# Autodesk Inventor assembly: climber assssssembly
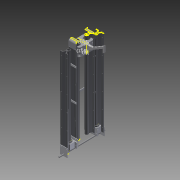
[picture p0: Inventor's stored thumbnail of the model, 180x180]
Saved by Autodesk Inventor 2013 (Build 170138000, 138)
## iProperties
Created: 2013-01-24
Part Number: climber assssssembly
Document SubType Name: Assembly
Designer: Arpan
Mass: 2447.33 g
Surface Area: 6955.59 cm^2
Volume: 1769.33 cm^3
Density: 1.3832 g/cm^3
Author: Arpan
## Documents named in this file (10)
- C:\Users\Arpan\Documents\GitHub\frc2013CAD\Climber\climber assssssembly.iam
- C:\Users\Arpan\Documents\GitHub\frc2013CAD\Climber\Shaft 26 inch.ipt
- C:\Users\Arpan\Documents\GitHub\frc2013CAD\Climber\Bearing Block long style.iam
- C:\Users\Arpan\Documents\GitHub\frc2013CAD\Climber\hook.ipt
- C:\Users\Arpan\Documents\GitHub\frc2013CAD\Climber\bearing block short style.iam
- C:\Users\Arpan\Documents\GitHub\frc2013CAD\Climber\endstop.ipt
- C:\Users\Arpan\Documents\GitHub\frc2013CAD\Climber\tie-together tier 1.ipt
- C:\Users\Arpan\Documents\GitHub\frc2013CAD\Climber\face mount.ipt
- C:\Users\Arpan\Documents\GitHub\frc2013CAD\Climber\arm mout.ipt
- C:\Users\Arpan\Documents\GitHub\frc2013CAD\Climber\shaft.ipt
## Components (19 placed, 9 different names)
1. Shaft 26 inch:1 — Angle:1, Mate:2, Angle:3, Flush:3, Mate:13, Flush:5, Mate:14, Flush:7, Mate:17, Mate:18, Mate:22, Mate:23, Mate:24, Angle:5
2. Shaft 26 inch:2 — Angle:1, Angle:2, Mate:3, Flush:3, Mate:15, Flush:6, Mate:16, Mate:19, Mate:20, Mate:21, Mate:28, Mate:29, Mate:30
3. Bearing Block long style:1 [sub-assembly] — Angle:2, Mate:3, Flush:2, Flush:4, Mate:4, Mate:8, Mate:9
4. Bearing Block long style:2 [sub-assembly] — Mate:2, Angle:3, Flush:2, Flush:4, Mate:4, Mate:5, Mate:6, Mate:7, Mate:10, Mate:11, Mate:12
5. hook:1 — Mate:5, Mate:6, Mate:7, Mate:10, Mate:11, Mate:12
6. hook:2 — Mate:8, Mate:9
7. bearing block short style:1 [sub-assembly] — Mate:25, Mate:26, Mate:27, Mate:36
8. bearing block short style:3 [sub-assembly] — Mate:31, Mate:32, Mate:33, Mate:34, Angle:4, Mate:35
9. endstop:1 — Mate:13, Flush:5, Mate:14
10. endstop:2 — Mate:15, Flush:6, Mate:16
11. tie-together tier 1:1 — Flush:7, Mate:17, Mate:18
12. tie-together tier 1:2 — Mate:19, Mate:20, Mate:21
13. face mount:1 — Mate:28, Mate:29, Mate:30, Mate:31, Mate:32, Mate:33
14. face mount:2 — Mate:22, Mate:23, Mate:24, Mate:25, Mate:26, Mate:27
15. Shaft 26 inch:3 — Mate:34, Angle:4, Mate:35, Mate:37, Mate:38, Mate:39, Flush:8
16. Shaft 26 inch:4 — Mate:36, Angle:5, Mate:44, Mate:45, Flush:8
17. arm mout:1 — Mate:37, Mate:38, Mate:39, Mate:43
18. shaft:1 — Mate:43
19. arm mout:2 — Mate:44, Mate:45
## Relationships (53: Mate 41, Flush 7, Angle 5)
- Angle:1 (180 deg): Shaft 26 inch:1 ↔ Shaft 26 inch:2
- Mate:2: Shaft 26 inch:1 ↔ Bearing Block long style:2
- Angle:2 (0 deg): Shaft 26 inch:2 ↔ Bearing Block long style:1
- Angle:3 (180 deg): Shaft 26 inch:1 ↔ Bearing Block long style:2
- Mate:3: Shaft 26 inch:2 ↔ Bearing Block long style:1
- Flush:2: Bearing Block long style:1 ↔ Bearing Block long style:2
- Flush:3: Shaft 26 inch:1 ↔ Shaft 26 inch:2
- Flush:4: Bearing Block long style:1 ↔ Bearing Block long style:2
- Mate:4 (12.7 mm): Bearing Block long style:1 ↔ Bearing Block long style:2
- Mate:5: Bearing Block long style:2 ↔ hook:1
- Mate:6: Bearing Block long style:2 ↔ hook:1
- Mate:7: Bearing Block long style:2 ↔ hook:1
- Mate:8: Bearing Block long style:1 ↔ hook:2
- Mate:9: Bearing Block long style:1 ↔ hook:2
- Mate:10: Bearing Block long style:2 ↔ hook:1
- Mate:11: Bearing Block long style:2 ↔ hook:1
- Mate:12: Bearing Block long style:2 ↔ hook:1
- Mate:13: Shaft 26 inch:1 ↔ endstop:1
- Flush:5: Shaft 26 inch:1 ↔ endstop:1
- Mate:14: Shaft 26 inch:1 ↔ endstop:1
- Mate:15: Shaft 26 inch:2 ↔ endstop:2
- Flush:6: Shaft 26 inch:2 ↔ endstop:2
- Mate:16: Shaft 26 inch:2 ↔ endstop:2
- Flush:7: Shaft 26 inch:1 ↔ tie-together tier 1:1
- Mate:17: Shaft 26 inch:1 ↔ tie-together tier 1:1
- Mate:18: Shaft 26 inch:1 ↔ tie-together tier 1:1
- Mate:19: Shaft 26 inch:2 ↔ tie-together tier 1:2
- Mate:20: Shaft 26 inch:2 ↔ tie-together tier 1:2
- Mate:21: Shaft 26 inch:2 ↔ tie-together tier 1:2
- Mate:22: Shaft 26 inch:1 ↔ face mount:2
- Mate:23: Shaft 26 inch:1 ↔ face mount:2
- Mate:24: Shaft 26 inch:1 ↔ face mount:2
- Mate:25: bearing block short style:1 ↔ face mount:2
- Mate:26: bearing block short style:1 ↔ face mount:2
- Mate:27: bearing block short style:1 ↔ face mount:2
- Mate:28: Shaft 26 inch:2 ↔ face mount:1
- Mate:29: Shaft 26 inch:2 ↔ face mount:1
- Mate:30: Shaft 26 inch:2 ↔ face mount:1
- Mate:31: bearing block short style:3 ↔ face mount:1
- Mate:32: bearing block short style:3 ↔ face mount:1
- Mate:33: bearing block short style:3 ↔ face mount:1
- Mate:34: bearing block short style:3 ↔ Shaft 26 inch:3
- Angle:4 (180 deg): bearing block short style:3 ↔ Shaft 26 inch:3
- Mate:35: bearing block short style:3 ↔ Shaft 26 inch:3
- Mate:36: bearing block short style:1 ↔ Shaft 26 inch:4
- Angle:5 (0 deg): Shaft 26 inch:1 ↔ Shaft 26 inch:4
- Mate:37: Shaft 26 inch:3 ↔ arm mout:1
- Mate:38: Shaft 26 inch:3 ↔ arm mout:1
- Mate:39: Shaft 26 inch:3 ↔ arm mout:1
- Mate:43: arm mout:1 ↔ shaft:1
- Mate:44: Shaft 26 inch:4 ↔ arm mout:2
- Mate:45: Shaft 26 inch:4 ↔ arm mout:2
- Flush:8: Shaft 26 inch:3 ↔ Shaft 26 inch:4
